# Autodesk Inventor assembly: Lift.03.00.00.00
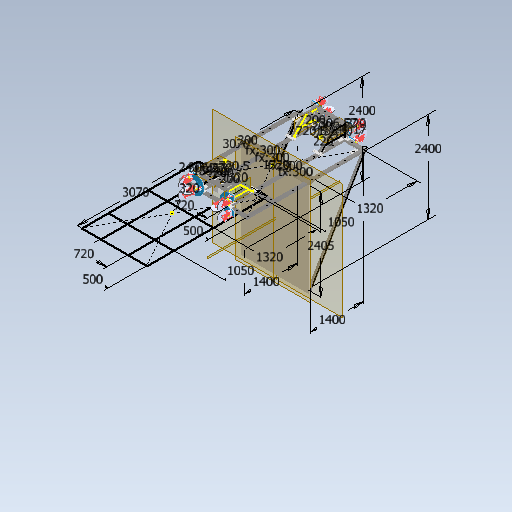
[picture p0: Inventor's stored thumbnail of the model, 512x512]
Saved by Autodesk Inventor 2021 (Build 250183000, 183)
## iProperties
Created: 2020-09-20
Part Number: Lift.03.00.00.00
Document SubType Name: Assembly
Designer: Kostya
Author: Kostya
## Documents named in this file (8)
- C:\Lift\Lift.03.00.00.00.iam
- C:\Lift\Lift.03.00.00.03.ipt
- C:\Lift\Lift.03.00.00.01.ipt
- C:\Lift\Lift.03.00.00.02.ipt
- C:\Lift\Lift.03.01.02.00.ipt
- C:\Lift\Lift.03.02.00.00.iam
- C:\Lift\Lift.03.01.00.00.iam
- C:\Lift\Роликовый узел.iam
## Components (14 placed, 7 different names)
1. Lift.03.00.00.03:1 — Совмещение:6, Совмещение:7
2. Lift.03.00.00.01:1 — Совмещение:3, Заподлицо:5, Заподлицо:6, Совмещение:6, Совмещение:7
3. Lift.03.00.00.02:1 — Совмещение:8, Заподлицо:14, Заподлицо:15, Заподлицо:21, Совмещение:11, Заподлицо:22, Заподлицо:26
4. Lift.03.01.02.00:1
5. Lift.03.00.00.02:2 — Совмещение:9, Заподлицо:16, Заподлицо:17, Совмещение:10, Заподлицо:19, Заподлицо:20, Заподлицо:31
6. Lift.03.02.00.00:1 [sub-assembly] — Совмещение:4, Заподлицо:10, Заподлицо:11, Заподлицо:18, Совмещение:13, Совмещение:15
7. Lift.03.02.00.00:2 [sub-assembly] — Совмещение:3, Заподлицо:5, Заподлицо:6, Совмещение:5, Заподлицо:12, Заподлицо:13, Заподлицо:14, Заподлицо:15, Заподлицо:16, Заподлицо:17, Заподлицо:18
8. Lift.03.01.00.00:1 [sub-assembly] — Заподлицо:7, Заподлицо:8, Заподлицо:9, Совмещение:4, Заподлицо:10, Заподлицо:11, Совмещение:5, Заподлицо:12, Заподлицо:13, Совмещение:8, Совмещение:9, Заподлицо:23
9. Роликовый узел:3 [sub-assembly] — Заподлицо:21, Совмещение:11, Заподлицо:22, Заподлицо:27
10. Роликовый узел:4 [sub-assembly] — Совмещение:10, Заподлицо:19, Заподлицо:20, Заподлицо:30
11. Lift.03.00.00.02:3 — Совмещение:13, Заподлицо:26, Заподлицо:27
12. Роликовый узел:5 [sub-assembly]
13. Lift.03.00.00.02:4 — Совмещение:15, Заподлицо:30, Заподлицо:31
14. Роликовый узел:6 [sub-assembly]
## Relationships (40: Flush 27, Mate 13)
- Совмещение:3 [Mate]: Lift.03.00.00.01:1 ↔ Lift.03.02.00.00:2
- Заподлицо:5 [Flush]: Lift.03.00.00.01:1 ↔ Lift.03.02.00.00:2
- Заподлицо:6 [Flush] (280.0325 mm): Lift.03.00.00.01:1 ↔ Lift.03.02.00.00:2
- Заподлицо:7 [Flush]: Lift.03.01.00.00:1
- Заподлицо:8 [Flush]: Lift.03.01.00.00:1
- Заподлицо:9 [Flush]: Lift.03.01.00.00:1
- Совмещение:4 [Mate]: Lift.03.02.00.00:1 ↔ Lift.03.01.00.00:1
- Заподлицо:10 [Flush]: Lift.03.02.00.00:1 ↔ Lift.03.01.00.00:1
- Заподлицо:11 [Flush]: Lift.03.02.00.00:1 ↔ Lift.03.01.00.00:1
- Совмещение:5 [Mate]: Lift.03.02.00.00:2 ↔ Lift.03.01.00.00:1
- Заподлицо:12 [Flush]: Lift.03.02.00.00:2 ↔ Lift.03.01.00.00:1
- Заподлицо:13 [Flush]: Lift.03.02.00.00:2 ↔ Lift.03.01.00.00:1
- Совмещение:6 [Mate]: Lift.03.00.00.03:1 ↔ Lift.03.00.00.01:1
- Совмещение:7 [Mate] (15 mm): Lift.03.00.00.03:1 ↔ Lift.03.00.00.01:1
- Совмещение:8 [Mate]: Lift.03.00.00.02:1 ↔ Lift.03.01.00.00:1
- Заподлицо:14 [Flush] (-5.5 mm): Lift.03.00.00.02:1 ↔ Lift.03.02.00.00:2
- Заподлицо:15 [Flush] (190 mm): Lift.03.00.00.02:1 ↔ Lift.03.02.00.00:2
- Совмещение:9 [Mate]: Lift.03.00.00.02:2 ↔ Lift.03.01.00.00:1
- Заподлицо:16 [Flush] (-5.5 mm): Lift.03.00.00.02:2 ↔ Lift.03.02.00.00:2
- Заподлицо:17 [Flush] (190 mm): Lift.03.00.00.02:2 ↔ Lift.03.02.00.00:2
- Заподлицо:18 [Flush]: Lift.03.02.00.00:1 ↔ Lift.03.02.00.00:2
- Совмещение:10 [Mate]: Lift.03.00.00.02:2 ↔ Роликовый узел:4
- Заподлицо:19 [Flush]: Lift.03.00.00.02:2 ↔ Роликовый узел:4
- Заподлицо:20 [Flush]: Lift.03.00.00.02:2 ↔ Роликовый узел:4
- Заподлицо:21 [Flush]: Lift.03.00.00.02:1 ↔ Роликовый узел:3
- Совмещение:11 [Mate]: Lift.03.00.00.02:1 ↔ Роликовый узел:3
- Заподлицо:22 [Flush]: Lift.03.00.00.02:1 ↔ Роликовый узел:3
- Заподлицо:23 [Flush] (-1575 mm): Lift.03.01.00.00:1
- [Flush]: Lift.03.00.00.02:3 ↔ Роликовый узел:5
- [Mate]: Lift.03.00.00.02:3 ↔ Роликовый узел:5
- [Flush]: Lift.03.00.00.02:3 ↔ Роликовый узел:5
- Совмещение:13 [Mate]: Lift.03.02.00.00:1 ↔ Lift.03.00.00.02:3
- Заподлицо:26 [Flush]: Lift.03.00.00.02:1 ↔ Lift.03.00.00.02:3
- Заподлицо:27 [Flush]: Роликовый узел:3 ↔ Lift.03.00.00.02:3
- [Flush]: Lift.03.00.00.02:4 ↔ Роликовый узел:6
- [Mate]: Lift.03.00.00.02:4 ↔ Роликовый узел:6
- [Flush]: Lift.03.00.00.02:4 ↔ Роликовый узел:6
- Совмещение:15 [Mate]: Lift.03.02.00.00:1 ↔ Lift.03.00.00.02:4
- Заподлицо:30 [Flush]: Роликовый узел:4 ↔ Lift.03.00.00.02:4
- Заподлицо:31 [Flush]: Lift.03.00.00.02:2 ↔ Lift.03.00.00.02:4
## Named parameters: d40_d30 = 0 mm, d41_d31 = 0 mm, d42_d32 = 0 mm, d46_d30 = 0 mm, d47_d31 = 0 mm, d48_d32 = 0 mm
